# Autodesk Inventor assembly: Project Assembly
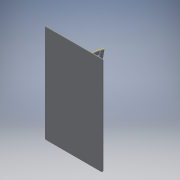
[picture p0: Inventor's stored thumbnail of the model, 180x180]
Saved by Autodesk Inventor 2019 (Build 230136000, 136)
## iProperties
Created: 2021-06-06
Part Number: Project Assembly
Document SubType Name: Assembly
Designer: micha
Author: micha
## Documents named in this file (17)
- D:\Files\ASU - Faculty of Engineering\Semester 10 - Spring 2021\Industrial Mechanisms and Robotics - MCT331\Four Bar Gripper Project\Project Assembly.iam
- D:\Files\ASU - Faculty of Engineering\Semester 10 - Spring 2021\Industrial Mechanisms and Robotics - MCT331\Four Bar Gripper Project\Base.ipt
- D:\Files\ASU - Faculty of Engineering\Semester 10 - Spring 2021\Industrial Mechanisms and Robotics - MCT331\Four Bar Gripper Project\NEMA 23 - 56mm.iam
- D:\Files\ASU - Faculty of Engineering\Semester 10 - Spring 2021\Industrial Mechanisms and Robotics - MCT331\Four Bar Gripper Project\nema23-mounting-L-bracket.ipt
- D:\Files\ASU - Faculty of Engineering\Semester 10 - Spring 2021\Industrial Mechanisms and Robotics - MCT331\Four Bar Gripper Project\Project Assembly\Design Accelerator\Spur Gears2.iam
- D:\Files\ASU - Faculty of Engineering\Semester 10 - Spring 2021\Industrial Mechanisms and Robotics - MCT331\Four Bar Gripper Project\Ruland_PCMR25-10-6-A.ipt
- D:\Files\ASU - Faculty of Engineering\Semester 10 - Spring 2021\Industrial Mechanisms and Robotics - MCT331\Four Bar Gripper Project\Small Gear Shaft.ipt
- D:\Files\ASU - Faculty of Engineering\Semester 10 - Spring 2021\Industrial Mechanisms and Robotics - MCT331\Four Bar Gripper Project\Large Gear Shaft.ipt
- D:\Files\ASU - Faculty of Engineering\Semester 10 - Spring 2021\Industrial Mechanisms and Robotics - MCT331\Four Bar Gripper Project\Bearing 10mm.ipt
- D:\Files\ASU - Faculty of Engineering\Semester 10 - Spring 2021\Industrial Mechanisms and Robotics - MCT331\Four Bar Gripper Project\Bearing Seats 10mm.ipt
- D:\Files\ASU - Faculty of Engineering\Semester 10 - Spring 2021\Industrial Mechanisms and Robotics - MCT331\Four Bar Gripper Project\ScaledAssembly.ipt
- D:\Files\ASU - Faculty of Engineering\Semester 10 - Spring 2021\Industrial Mechanisms and Robotics - MCT331\Four Bar Gripper Project\Fourbar-Crank.ipt
- D:\Files\ASU - Faculty of Engineering\Semester 10 - Spring 2021\Industrial Mechanisms and Robotics - MCT331\Four Bar Gripper Project\Fourbar-Coupler.ipt
- D:\Files\ASU - Faculty of Engineering\Semester 10 - Spring 2021\Industrial Mechanisms and Robotics - MCT331\Four Bar Gripper Project\Fourbar-Rocker.ipt
- C:\Users\micha\OneDrive\Documents\Inventor\Content Center Files\R2019\en-US\Nut GB_T 13807.3-1992 Type G\Nut GB_T 13807.3-1992 Type G M12.ipt
- D:\Files\ASU - Faculty of Engineering\Semester 10 - Spring 2021\Industrial Mechanisms and Robotics - MCT331\Four Bar Gripper Project\Rocker Base Shaft.ipt
- D:\Files\ASU - Faculty of Engineering\Semester 10 - Spring 2021\Industrial Mechanisms and Robotics - MCT331\Four Bar Gripper Project\Bearing Seats 10mm (Short).ipt
## Components (28 placed, 16 different names)
1. Base:1 — Mate:2, Angle:2, Flush:1, Flush:2, Angle:4, Mate:21, Mate:26, Angle:5, Angle:6, Angle:7, Angle:8, Mate:70, Mate:71, Mate:72, Mate:76
2. NEMA 23 - 56mm:1 [sub-assembly] — Mate:1, Mate:3, Angle:1, Mate:4, Mate:5, Mate:43
3. nema23-mounting-L-bracket:1 — Mate:1, Mate:2, Mate:3, Angle:1, Angle:2, Flush:1, Flush:2
4. Spur Gears:1 [sub-assembly] — Mate:4, Flush:3, Mate:16, Mate:28, Mate:45, Mate:48, Mate:52, Mate:54
5. Ruland_PCMR25-10-6-A:1 — Mate:5, Mate:43, Mate:55
6. Small Gear Shaft:1 — Mate:48, Mate:49, Mate:50, Mate:51, Mate:53, Mate:55, Mate:56, Mate:57
7. Large Gear Shaft:1 — Flush:3, Mate:16, Mate:17, Mate:18, Mate:19, Mate:20, Mate:29, Mate:44, Mate:46, Angle:8, Mate:69
8. Bearing 10mm:1 — Mate:17, Mate:18, Angle:4, Flush:4, Mate:22, Mate:23, Mate:24
9. Bearing 10mm:2 — Mate:19, Mate:20, Flush:4, Mate:25, Mate:27, Flush:6
10. Bearing Seats 10mm:1 — Mate:21, Mate:22, Mate:23, Mate:24
11. Bearing Seats 10mm:2 — Mate:25, Mate:26, Mate:27
12. ScaledAssembly:1 — Mate:34, Mate:35, Flush:5
13. Fourbar-Crank:1 — Mate:28, Mate:29, Mate:30, Mate:31, Mate:47
14. Fourbar-Coupler:1 — Mate:30, Mate:31, Mate:32, Mate:58
15. Fourbar-Rocker:1 — Mate:32, Mate:34, Mate:35, Flush:5, Mate:58, Mate:59, Mate:64, Mate:66, Mate:68
16. Nut GB/T 13807.3-1992 Type G M12:1 — Mate:44, Mate:45
17. Nut GB/T 13807.3-1992 Type G M12:2 — Mate:46, Mate:47
18. Bearing 10mm:3 — Mate:49, Mate:50, Angle:5, Flush:6, Mate:75, Mate:77
19. Nut GB/T 13807.3-1992 Type G M12:3 — Mate:51, Mate:52
20. Nut GB/T 13807.3-1992 Type G M12:4 — Mate:53, Mate:54
21. Bearing 10mm:4 — Mate:56, Mate:57, Angle:6, Mate:73, Mate:74
22. Rocker Base Shaft:1 — Mate:59, Mate:60, Mate:61, Mate:62, Mate:63, Mate:64, Mate:65, Mate:67, Angle:7, Mate:69
23. Bearing 10mm:5 — Mate:60, Mate:63, Mate:71
24. Bearing 10mm:6 — Mate:61, Mate:62, Mate:70
25. Nut GB/T 13807.3-1992 Type G M12:5 — Mate:65, Mate:66
26. Nut GB/T 13807.3-1992 Type G M12:6 — Mate:67, Mate:68
27. Bearing Seats 10mm (Short):1 — Mate:72, Mate:73, Mate:74
28. Bearing Seats 10mm (Short):2 — Mate:75, Mate:76, Mate:77
## Relationships (72: Mate 59, Angle 7, Flush 6)
- Mate:1: NEMA 23 - 56mm:1 ↔ nema23-mounting-L-bracket:1
- Mate:2: Base:1 ↔ nema23-mounting-L-bracket:1
- Mate:3: NEMA 23 - 56mm:1 ↔ nema23-mounting-L-bracket:1
- Angle:1 (0 deg): NEMA 23 - 56mm:1 ↔ nema23-mounting-L-bracket:1
- Angle:2 (0 deg): Base:1 ↔ nema23-mounting-L-bracket:1
- Mate:4: NEMA 23 - 56mm:1 ↔ Spur Gears:1
- Flush:1 (50 mm): Base:1 ↔ nema23-mounting-L-bracket:1
- Mate:5: NEMA 23 - 56mm:1 ↔ Ruland_PCMR25-10-6-A:1
- Flush:2 (80 mm): Base:1 ↔ nema23-mounting-L-bracket:1
- Flush:3 (5 mm): Spur Gears:1 ↔ Large Gear Shaft:1
- Mate:16: Spur Gears:1 ↔ Large Gear Shaft:1
- Mate:17: Large Gear Shaft:1 ↔ Bearing 10mm:1
- Mate:18: Large Gear Shaft:1 ↔ Bearing 10mm:1
- Angle:4 (180 deg): Base:1 ↔ Bearing 10mm:1
- Mate:19: Large Gear Shaft:1 ↔ Bearing 10mm:2
- Mate:20: Large Gear Shaft:1 ↔ Bearing 10mm:2
- Flush:4: Bearing 10mm:1 ↔ Bearing 10mm:2
- Mate:21: Base:1 ↔ Bearing Seats 10mm:1
- Mate:22: Bearing 10mm:1 ↔ Bearing Seats 10mm:1
- Mate:23: Bearing 10mm:1 ↔ Bearing Seats 10mm:1
- Mate:24: Bearing 10mm:1 ↔ Bearing Seats 10mm:1
- Mate:25: Bearing 10mm:2 ↔ Bearing Seats 10mm:2
- Mate:26: Base:1 ↔ Bearing Seats 10mm:2
- Mate:27: Bearing 10mm:2 ↔ Bearing Seats 10mm:2
- Mate:28: Spur Gears:1 ↔ Fourbar-Crank:1
- Mate:29: Large Gear Shaft:1 ↔ Fourbar-Crank:1
- Mate:30: Fourbar-Crank:1 ↔ Fourbar-Coupler:1
- Mate:31: Fourbar-Crank:1 ↔ Fourbar-Coupler:1
- Mate:32: Fourbar-Coupler:1 ↔ Fourbar-Rocker:1
- Mate:34: ScaledAssembly:1 ↔ Fourbar-Rocker:1
- Mate:35 (-100 mm): ScaledAssembly:1 ↔ Fourbar-Rocker:1
- Flush:5: ScaledAssembly:1 ↔ Fourbar-Rocker:1
- Mate:43 (-7 mm): NEMA 23 - 56mm:1 ↔ Ruland_PCMR25-10-6-A:1
- Mate:44: Large Gear Shaft:1 ↔ Nut GB/T 13807.3-1992 Type G M12:1
- Mate:45: Spur Gears:1 ↔ Nut GB/T 13807.3-1992 Type G M12:1
- Mate:46: Large Gear Shaft:1 ↔ Nut GB/T 13807.3-1992 Type G M12:2
- Mate:47: Fourbar-Crank:1 ↔ Nut GB/T 13807.3-1992 Type G M12:2
- Mate:48: Spur Gears:1 ↔ Small Gear Shaft:1
- Mate:49: Small Gear Shaft:1 ↔ Bearing 10mm:3
- Mate:50: Small Gear Shaft:1 ↔ Bearing 10mm:3
- Angle:5 (180 deg): Base:1 ↔ Bearing 10mm:3
- Flush:6: Bearing 10mm:2 ↔ Bearing 10mm:3
- Mate:51: Small Gear Shaft:1 ↔ Nut GB/T 13807.3-1992 Type G M12:3
- Mate:52: Spur Gears:1 ↔ Nut GB/T 13807.3-1992 Type G M12:3
- Mate:53: Small Gear Shaft:1 ↔ Nut GB/T 13807.3-1992 Type G M12:4
- Mate:54: Spur Gears:1 ↔ Nut GB/T 13807.3-1992 Type G M12:4
- Mate:55 (-12 mm): Ruland_PCMR25-10-6-A:1 ↔ Small Gear Shaft:1
- Mate:56: Small Gear Shaft:1 ↔ Bearing 10mm:4
- Mate:57: Small Gear Shaft:1 ↔ Bearing 10mm:4
- Angle:6 (180 deg): Base:1 ↔ Bearing 10mm:4
- Mate:58: Fourbar-Coupler:1 ↔ Fourbar-Rocker:1
- Mate:59: Fourbar-Rocker:1 ↔ Rocker Base Shaft:1
- Mate:60: Rocker Base Shaft:1 ↔ Bearing 10mm:5
- Mate:61: Rocker Base Shaft:1 ↔ Bearing 10mm:6
- Mate:62: Rocker Base Shaft:1 ↔ Bearing 10mm:6
- Mate:63: Rocker Base Shaft:1 ↔ Bearing 10mm:5
- Mate:64 (-6 mm): Fourbar-Rocker:1 ↔ Rocker Base Shaft:1
- Mate:65: Rocker Base Shaft:1 ↔ Nut GB/T 13807.3-1992 Type G M12:5
- Mate:66: Fourbar-Rocker:1 ↔ Nut GB/T 13807.3-1992 Type G M12:5
- Mate:67: Rocker Base Shaft:1 ↔ Nut GB/T 13807.3-1992 Type G M12:6
- Mate:68: Fourbar-Rocker:1 ↔ Nut GB/T 13807.3-1992 Type G M12:6
- Angle:7 (0 deg): Base:1 ↔ Rocker Base Shaft:1
- Angle:8 (0 deg): Base:1 ↔ Large Gear Shaft:1
- Mate:69 (-310 mm): Large Gear Shaft:1 ↔ Rocker Base Shaft:1
- Mate:70: Base:1 ↔ Bearing 10mm:6
- Mate:71: Base:1 ↔ Bearing 10mm:5
- Mate:72: Base:1 ↔ Bearing Seats 10mm (Short):1
- Mate:73: Bearing 10mm:4 ↔ Bearing Seats 10mm (Short):1
- Mate:74: Bearing 10mm:4 ↔ Bearing Seats 10mm (Short):1
- Mate:75: Bearing 10mm:3 ↔ Bearing Seats 10mm (Short):2
- Mate:76: Base:1 ↔ Bearing Seats 10mm (Short):2
- Mate:77: Bearing 10mm:3 ↔ Bearing Seats 10mm (Short):2
